# Autodesk Inventor assembly: main_sumec_assembly
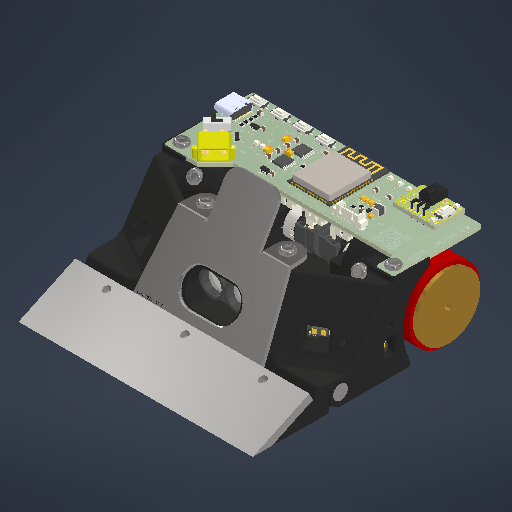
[picture p0: Inventor's stored thumbnail of the model, 512x512]
Saved by Autodesk Inventor 2025.3 (Build 293356000, 356)
## iProperties
Created: 2025-03-23
Part Number: main_sumec_assembly
Document SubType Name: Assembly
Designer: Simak
Author: Simak
## Documents named in this file (19)
- C:\_desktop\Sumec-MiniSumo-MECH\!main_sumec_assembly.iam
- C:\_desktop\Sumec-MiniSumo-MECH\3D_printed\body-main.ipt
- C:\_desktop\Sumec-MiniSumo-MECH\3D_printed\body-front.ipt
- C:\_desktop\Sumec-MiniSumo-MECH\3D_printed\body-motor_comparment.ipt
- C:\_desktop\Sumec-MiniSumo-MECH\3D_printed\motor_C_clamp.ipt
- C:\_desktop\Sumec-MiniSumo-MECH\electronics\AssemBeneWake TF-LUNA.ipt
- C:\_desktop\Sumec-MiniSumo-MECH\electronics\pololu_12v_650rpm-cb-enc-side-con.ipt
- C:\_desktop\Sumec-MiniSumo-MECH\electronics\pololu-digital-distance-sensor-irs17a.ipt
- C:\_desktop\Sumec-MiniSumo-MECH\electronics\PCBs\main board\SUMEC_MK_V .iam
- C:\_desktop\Sumec-MiniSumo-MECH\machined\lowerRamp.ipt
- C:\_desktop\Sumec-MiniSumo-MECH\machined\wheelGen2.ipt
- C:\_desktop\Sumec-MiniSumo-MECH\electronics\PCBs\QRE MiniBoards\QRE_MiniBoardV2.iam
- C:\_desktop\Sumec-MiniSumo-MECH\other\bublegum.ipt
- C:\_desktop\Sumec-MiniSumo-MECH\machined\trubicka.ipt
- C:\_desktop\Sumec-MiniSumo-MECH\electronics\SUMEC_MK_IV.iam
- C:\_desktop\Sumec-MiniSumo-MECH\fasteners\screws\M3_kuzel_torx\torx_socket_countersunk_flat_head_M3x06.ipt
- C:\_desktop\Sumec-MiniSumo-MECH\fasteners\screws\M3_koule_torx\torx_socket_button_head_M3x08.ipt
- C:\_desktop\Sumec-MiniSumo-MECH\fasteners\screws\M3_valec_torx\torx_socket_cylindrical_head_M3x25.ipt
- C:\_desktop\Sumec-MiniSumo-MECH\machined\MK_5_rust_helma1.ipt
## Components (34 placed, 18 different names)
1. body-main:1 — Vložit:1, Vložit:2, Vložit:5, Proti sobě:13, Vložit:6, Proti sobě:14, Vložit:22, Vložit:23, Úhel:1, lock
2. body-front:1 — Vložit:1, Proti sobě:6, Stejný směr:3, Vložit:3, Vložit:4, Proti sobě:7, Vložit:7, Proti sobě:8, Vložit:10, Proti sobě:15, Proti sobě:16, Proti sobě:17, Vložit:17, Vložit:18, Vložit:19, Vložit:20, Vložit:21, Proti sobě:18, Stejný směr:8, lock, Stejný směr:11, Proti sobě:22
3. body-motor_comparment:1 — Vložit:2, Proti sobě:1, Proti sobě:2, Proti sobě:4, Stejný směr:2, Stejný směr:6, Proti sobě:10, Stejný směr:7, Proti sobě:12, Vložit:16, Úhel:1, Stejný směr:9, Stejný směr:10, Proti sobě:20, Proti sobě:21
4. motor_C_clamp:1 — Stejný směr:6, Proti sobě:10, Stejný směr:9
5. AssemBeneWake TF-LUNA:1 — Proti sobě:6, Stejný směr:3, Vložit:3
6. pololu_12v_650rpm-cb-enc-side-con:1 — Proti sobě:1, Proti sobě:2, Vložit:13, Proti sobě:20
7. pololu-digital-distance-sensor-irs17a:1 — Vložit:4, Proti sobě:7
8. pololu_12v_650rpm-cb-enc-side-con:2 — Proti sobě:4, Stejný směr:2, Vložit:12, Proti sobě:21
9. pololu-digital-distance-sensor-irs17a:2 — Vložit:7, Proti sobě:8
10. pololu-digital-distance-sensor-irs17a:3 — Vložit:5, Proti sobě:13
11. pololu-digital-distance-sensor-irs17a:4 — Vložit:6, Proti sobě:14
12. motor_C_clamp:2 — Stejný směr:7, Proti sobě:12, Stejný směr:10
13. SUMEC_MK_V :1 [sub-assembly]
14. lowerRamp:1 — Vložit:10, Stejný směr:11
15. wheelGen2:1 — Vložit:13, Vložit:15
16. QRE_MiniBoardV2:1 [sub-assembly]
17. wheelGen2:2 — Vložit:12, Vložit:14
18. bublegum:1 — Vložit:14
19. bublegum:2 — Vložit:15
20. trubicka:1 — Vložit:16, Vložit:24
21. SUMEC_MK_IV:1 [sub-assembly] — Proti sobě:15, Proti sobě:16, Proti sobě:17, Vložit:25, Vložit:26
22. torx_socket_countersunk_flat_head_M3x06:1 — Vložit:21
23. torx_socket_countersunk_flat_head_M3x06:2 — Vložit:19
24. torx_socket_countersunk_flat_head_M3x06:3 — Vložit:20
25. torx_socket_button_head_M3x08:1 — Vložit:18
26. torx_socket_button_head_M3x08:2 — Vložit:17
27. torx_socket_countersunk_flat_head_M3x06:4 — Vložit:23
28. torx_socket_countersunk_flat_head_M3x06:5 — Vložit:22
29. torx_socket_cylindrical_head_M3x25:1 — Vložit:24
30. torx_socket_button_head_M3x08:3 — Vložit:25
31. torx_socket_button_head_M3x08:4 — Vložit:26
32. MK_5_rust_helma1:1 — Proti sobě:18, Stejný směr:8, Vložit:27, Vložit:28, Proti sobě:22
33. torx_socket_button_head_M3x08:5 — Vložit:27
34. torx_socket_button_head_M3x08:6 — Vložit:28
## Relationships (52: Insert 25, Mate 17, Flush 8, Angle 2)
- Vložit:1 [Insert]: body-main:1 ↔ body-front:1
- Vložit:2 [Insert] (0.75 mm): body-main:1 ↔ body-motor_comparment:1
- Proti sobě:1 [Mate]: body-motor_comparment:1 ↔ pololu_12v_650rpm-cb-enc-side-con:1
- Proti sobě:2 [Mate]: body-motor_comparment:1 ↔ pololu_12v_650rpm-cb-enc-side-con:1
- Proti sobě:4 [Mate]: body-motor_comparment:1 ↔ pololu_12v_650rpm-cb-enc-side-con:2
- Stejný směr:2 [Flush]: body-motor_comparment:1 ↔ pololu_12v_650rpm-cb-enc-side-con:2
- Proti sobě:6 [Mate]: body-front:1 ↔ AssemBeneWake TF-LUNA:1
- Stejný směr:3 [Flush]: body-front:1 ↔ AssemBeneWake TF-LUNA:1
- Vložit:3 [Insert]: body-front:1 ↔ AssemBeneWake TF-LUNA:1
- Vložit:4 [Insert]: body-front:1 ↔ pololu-digital-distance-sensor-irs17a:1
- Proti sobě:7 [Mate]: body-front:1 ↔ pololu-digital-distance-sensor-irs17a:1
- Vložit:5 [Insert]: body-main:1 ↔ pololu-digital-distance-sensor-irs17a:3
- Proti sobě:13 [Mate]: body-main:1 ↔ pololu-digital-distance-sensor-irs17a:3
- Vložit:6 [Insert]: body-main:1 ↔ pololu-digital-distance-sensor-irs17a:4
- Proti sobě:14 [Mate]: body-main:1 ↔ pololu-digital-distance-sensor-irs17a:4
- Vložit:7 [Insert]: body-front:1 ↔ pololu-digital-distance-sensor-irs17a:2
- Proti sobě:8 [Mate]: body-front:1 ↔ pololu-digital-distance-sensor-irs17a:2
- Stejný směr:6 [Flush]: body-motor_comparment:1 ↔ motor_C_clamp:1
- Proti sobě:10 [Mate] (1 mm): body-motor_comparment:1 ↔ motor_C_clamp:1
- Stejný směr:7 [Flush]: body-motor_comparment:1 ↔ motor_C_clamp:2
- Proti sobě:12 [Mate] (1 mm): body-motor_comparment:1 ↔ motor_C_clamp:2
- Vložit:10 [Insert]: body-front:1 ↔ lowerRamp:1
- Vložit:12 [Insert]: pololu_12v_650rpm-cb-enc-side-con:2 ↔ wheelGen2:2
- Vložit:13 [Insert]: pololu_12v_650rpm-cb-enc-side-con:1 ↔ wheelGen2:1
- Vložit:14 [Insert]: wheelGen2:2 ↔ bublegum:1
- Vložit:15 [Insert]: wheelGen2:1 ↔ bublegum:2
- Vložit:16 [Insert]: body-motor_comparment:1 ↔ trubicka:1
- Proti sobě:15 [Mate]: body-front:1 ↔ SUMEC_MK_IV:1
- Proti sobě:16 [Mate]: body-front:1 ↔ SUMEC_MK_IV:1
- Proti sobě:17 [Mate]: body-front:1 ↔ SUMEC_MK_IV:1
- Vložit:17 [Insert]: body-front:1 ↔ torx_socket_button_head_M3x08:2
- Vložit:18 [Insert]: body-front:1 ↔ torx_socket_button_head_M3x08:1
- Vložit:19 [Insert]: body-front:1 ↔ torx_socket_countersunk_flat_head_M3x06:2
- Vložit:20 [Insert]: body-front:1 ↔ torx_socket_countersunk_flat_head_M3x06:3
- Vložit:21 [Insert]: body-front:1 ↔ torx_socket_countersunk_flat_head_M3x06:1
- Vložit:22 [Insert]: body-main:1 ↔ torx_socket_countersunk_flat_head_M3x06:5
- Vložit:23 [Insert]: body-main:1 ↔ torx_socket_countersunk_flat_head_M3x06:4
- Vložit:24 [Insert]: trubicka:1 ↔ torx_socket_cylindrical_head_M3x25:1
- Vložit:25 [Insert]: SUMEC_MK_IV:1 ↔ torx_socket_button_head_M3x08:3
- Vložit:26 [Insert]: SUMEC_MK_IV:1 ↔ torx_socket_button_head_M3x08:4
- Proti sobě:18 [Mate]: body-front:1 ↔ MK_5_rust_helma1:1
- Stejný směr:8 [Flush]: body-front:1 ↔ MK_5_rust_helma1:1
- Vložit:27 [Insert]: MK_5_rust_helma1:1 ↔ torx_socket_button_head_M3x08:5
- Vložit:28 [Insert]: MK_5_rust_helma1:1 ↔ torx_socket_button_head_M3x08:6
- Úhel:1 [Angle] (90 deg): body-main:1 ↔ body-motor_comparment:1
- Stejný směr:9 [Flush]: body-motor_comparment:1 ↔ motor_C_clamp:1
- Stejný směr:10 [Flush]: body-motor_comparment:1 ↔ motor_C_clamp:2
- Proti sobě:20 [Mate]: body-motor_comparment:1 ↔ pololu_12v_650rpm-cb-enc-side-con:1
- Proti sobě:21 [Mate]: body-motor_comparment:1 ↔ pololu_12v_650rpm-cb-enc-side-con:2
- lock [Angle] (0 deg): body-main:1 ↔ body-front:1
- Stejný směr:11 [Flush]: body-front:1 ↔ lowerRamp:1
- Proti sobě:22 [Mate]: body-front:1 ↔ MK_5_rust_helma1:1
